# Autodesk Inventor assembly: Righter
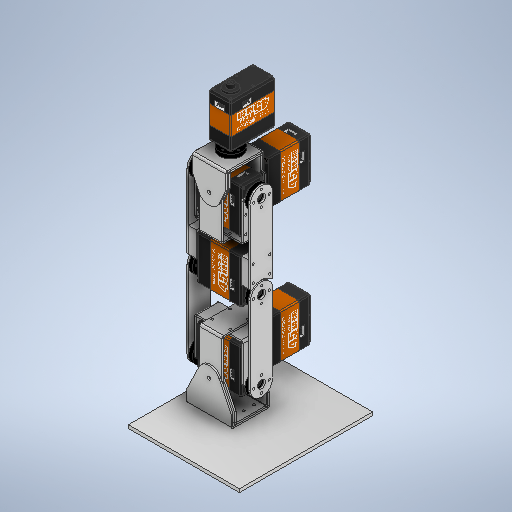
[picture p0: Inventor's stored thumbnail of the model, 512x512]
Saved by Autodesk Inventor 2025.2 (Build 292293000, 293)
## iProperties
Created: 2025-07-23
Part Number: Righter
Document SubType Name: Assembly
Designer: User
Author: User
## Documents named in this file (19)
- C:\Users\User\Documents\The Maverick's Files\College 3-3\로보인 프로젝트\RHp_Humanoid_ver1\Part\Frame\Leg\Righter.iam
- C:\Users\User\Documents\The Maverick's Files\College 3-3\로보인 프로젝트\RHp_Humanoid_ver1\Part\HTD-45H, Horn\HTD-45H\HTD-45H.iam
- C:\Users\User\Documents\The Maverick's Files\College 3-3\로보인 프로젝트\RHp_Humanoid_ver1\Part\HTD-45H, Horn\Horn\Bottom Horn.ipt
- C:\Users\User\Documents\The Maverick's Files\College 3-3\로보인 프로젝트\RHp_Humanoid_ver1\Part\HTD-45H, Horn\Horn\Top Horn.ipt
- C:\Users\User\Documents\The Maverick's Files\College 3-3\로보인 프로젝트\RHp_Humanoid_ver1\Part\Frame\Leg\axis_7_top_frame.ipt
- C:\Users\User\Documents\The Maverick's Files\College 3-3\로보인 프로젝트\RHp_Humanoid_ver1\Part\Frame\Leg\axis_9_bottom_frame.ipt
- C:\Users\User\Documents\The Maverick's Files\College 3-3\로보인 프로젝트\RHp_Humanoid_ver1\Part\Frame\Leg\partpart.ipt
- C:\Users\User\Documents\The Maverick's Files\College 3-3\로보인 프로젝트\RHp_Humanoid_ver1\Part\Frame\Leg\axis_8_bottom_frame.ipt
- C:\Users\User\Documents\The Maverick's Files\College 3-3\로보인 프로젝트\RHp_Humanoid_ver1\Part\Frame\Leg\axis_8_10_connector_frame_non_powered.ipt
- C:\Users\User\Documents\The Maverick's Files\College 3-3\로보인 프로젝트\RHp_Humanoid_ver1\Part\Frame\Leg\axis_8_10_connector_frame_powered.ipt
- C:\Users\User\Documents\The Maverick's Files\College 3-3\로보인 프로젝트\RHp_Humanoid_ver1\Part\Frame\Leg\3D_printed_part_non_powered.ipt
- C:\Users\User\Documents\The Maverick's Files\College 3-3\로보인 프로젝트\RHp_Humanoid_ver1\Part\Frame\Leg\3D_printed_part_powered.ipt
- C:\Users\User\Documents\The Maverick's Files\College 3-3\로보인 프로젝트\RHp_Humanoid_ver1\Part\Frame\Leg\axis_10_11-connector_frame_non_powered.ipt
- C:\Users\User\Documents\The Maverick's Files\College 3-3\로보인 프로젝트\RHp_Humanoid_ver1\Part\Frame\Leg\axis_10_11-connector_frame_powered.ipt
- C:\Users\User\Documents\The Maverick's Files\College 3-3\로보인 프로젝트\RHp_Humanoid_ver1\Part\Frame\Leg\axis_11_top_frame.ipt
- C:\Users\User\Documents\The Maverick's Files\College 3-3\로보인 프로젝트\RHp_Humanoid_ver1\Part\Frame\Leg\axis_12_top_frame.ipt
- C:\Users\User\Documents\The Maverick's Files\College 3-3\로보인 프로젝트\RHp_Humanoid_ver1\Part\Frame\Leg\axis_12_bottom_frame(top).ipt
- C:\Users\User\Documents\The Maverick's Files\College 3-3\로보인 프로젝트\RHp_Humanoid_ver1\Part\Frame\Leg\axis_12_supplement_frame.ipt
- C:\Users\User\Documents\The Maverick's Files\College 3-3\로보인 프로젝트\RHp_Humanoid_ver1\Part\Frame\Leg\axis_12_bottom_frame(bottom).ipt
## Components (30 placed, 18 different names)
1. HTD-45H:1 [sub-assembly] — Rotational:1
2. HTD-45H:2 [sub-assembly] — Rotational:2, Rigid:5
3. HTD-45H:3 [sub-assembly] — Rigid:6, Rotational:3, Rotational:4
4. HTD-45H:4 [sub-assembly] — Rigid:12, Rigid:13, Rotational:5, Rotational:6
5. HTD-45H:5 [sub-assembly] — Rigid:16, Rotational:7, Rotational:8
6. HTD-45H:6 [sub-assembly] — Rotational:9, Rigid:19
7. Bottom Horn:3 — Rotational:3, Rigid:8
8. Bottom Horn:4 — Rotational:5, Rigid:15
9. Bottom Horn:5 — Rotational:8, Rigid:18
10. Top Horn:1 — Rotational:1, Rigid:1
11. Top Horn:2 — Rotational:2, Rigid:2
12. Top Horn:3 — Rotational:4, Rigid:9
13. Top Horn:4 — Rotational:6, Rigid:14
14. Top Horn:5 — Rotational:7, Rigid:17
15. Top Horn:6 — Rotational:9, Rigid:20
16. axis_7_top_frame:1 — Rigid:1, Rigid:2, Rigid:4
17. axis_9_bottom_frame:1 — Rigid:5, Rigid:7
18. partpart:1 — Rigid:4
19. axis_8_bottom_frame:1 — Rigid:6, Rigid:7
20. axis_8_10_connector_frame_non_powered:1 — Rigid:8, Rigid:10
21. axis_8_10_connector_frame_powered:1 — Rigid:9, Rigid:11
22. 3D_printed_part_non_powered:1 — Rigid:10, Rigid:13
23. 3D_printed_part_powered:1 — Rigid:11, Rigid:12
24. axis_10_11-connector_frame_non_powered:1 — Rigid:15, Rigid:18
25. axis_10_11-connector_frame_powered:1 — Rigid:14, Rigid:17
26. axis_11_top_frame:1 — Rigid:16, Rigid:21
27. axis_12_top_frame:1 — Rigid:19, Rigid:21
28. axis_12_bottom_frame(top):1 — Rigid:20, Rigid:22, Rigid:23
29. axis_12_supplement_frame:1 — Rigid:22
30. axis_12_bottom_frame(bottom):1 — Rigid:23
## Relationships (31: WeldJoint 22, RevoluteJoint 9)
- Rotational:1 [RevoluteJoint]: HTD-45H:1 ↔ Top Horn:1
- Rigid:1 [WeldJoint]: Top Horn:1 ↔ axis_7_top_frame:1
- Rotational:2 [RevoluteJoint]: HTD-45H:2 ↔ Top Horn:2
- Rigid:2 [WeldJoint]: Top Horn:2 ↔ axis_7_top_frame:1
- Rigid:4 [WeldJoint]: axis_7_top_frame:1 ↔ partpart:1
- Rigid:5 [WeldJoint]: HTD-45H:2 ↔ axis_9_bottom_frame:1
- Rigid:6 [WeldJoint]: HTD-45H:3 ↔ axis_8_bottom_frame:1
- Rigid:7 [WeldJoint]: axis_9_bottom_frame:1 ↔ axis_8_bottom_frame:1
- Rotational:3 [RevoluteJoint]: HTD-45H:3 ↔ Bottom Horn:3
- Rotational:4 [RevoluteJoint]: HTD-45H:3 ↔ Top Horn:3
- Rigid:8 [WeldJoint]: Bottom Horn:3 ↔ axis_8_10_connector_frame_non_powered:1
- Rigid:9 [WeldJoint]: Top Horn:3 ↔ axis_8_10_connector_frame_powered:1
- Rigid:10 [WeldJoint]: axis_8_10_connector_frame_non_powered:1 ↔ 3D_printed_part_non_powered:1
- Rigid:11 [WeldJoint]: axis_8_10_connector_frame_powered:1 ↔ 3D_printed_part_powered:1
- Rigid:12 [WeldJoint]: HTD-45H:4 ↔ 3D_printed_part_powered:1
- Rigid:13 [WeldJoint]: HTD-45H:4 ↔ 3D_printed_part_non_powered:1
- Rotational:5 [RevoluteJoint]: HTD-45H:4 ↔ Bottom Horn:4
- Rotational:6 [RevoluteJoint]: HTD-45H:4 ↔ Top Horn:4
- Rigid:15 [WeldJoint]: Bottom Horn:4 ↔ axis_10_11-connector_frame_non_powered:1
- Rigid:14 [WeldJoint]: Top Horn:4 ↔ axis_10_11-connector_frame_powered:1
- Rigid:16 [WeldJoint]: HTD-45H:5 ↔ axis_11_top_frame:1
- Rotational:7 [RevoluteJoint]: HTD-45H:5 ↔ Top Horn:5
- Rotational:8 [RevoluteJoint]: HTD-45H:5 ↔ Bottom Horn:5
- Rigid:17 [WeldJoint]: Top Horn:5 ↔ axis_10_11-connector_frame_powered:1
- Rigid:18 [WeldJoint]: Bottom Horn:5 ↔ axis_10_11-connector_frame_non_powered:1
- Rotational:9 [RevoluteJoint]: HTD-45H:6 ↔ Top Horn:6
- Rigid:19 [WeldJoint]: HTD-45H:6 ↔ axis_12_top_frame:1
- Rigid:20 [WeldJoint]: Top Horn:6 ↔ axis_12_bottom_frame(top):1
- Rigid:21 [WeldJoint]: axis_11_top_frame:1 ↔ axis_12_top_frame:1
- Rigid:22 [WeldJoint]: axis_12_bottom_frame(top):1 ↔ axis_12_supplement_frame:1
- Rigid:23 [WeldJoint]: axis_12_bottom_frame(top):1 ↔ axis_12_bottom_frame(bottom):1
